# Autodesk Inventor assembly: Ensamblaje del tambor con sis. Lebus
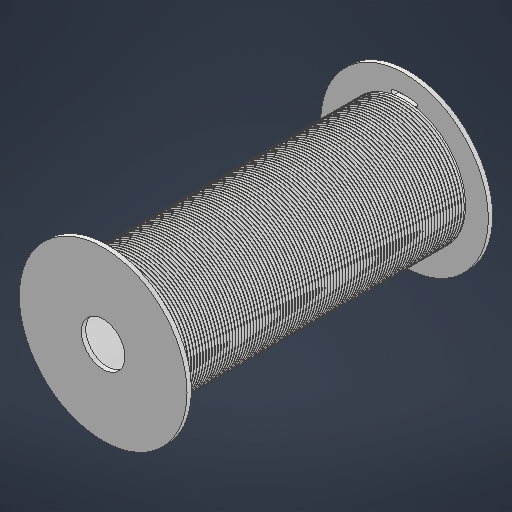
[picture p0: Inventor's stored thumbnail of the model, 512x512]
Saved by Autodesk Inventor 2026 (Build 300175050, 175E)
## iProperties
Created: 2025-07-06
Part Number: Ensamblaje del tambor con sis. Lebus
Document SubType Name: Conjunto soldado
Designer: Daniel Rodriguez
Weld Material: Genérico
Author: Daniel Rodriguez
## Documents named in this file (5)
- C:\Users\Daniel Rodriguez\Downloads\winch-drum-welding-assembly\Nuestro Winch\Sistema LEBUS\Ensamblaje del tambor con sis. Lebus.iam
- C:\Users\Daniel Rodriguez\Downloads\winch-drum-welding-assembly\Nuestro Winch\Sistema LEBUS\Tambor liso (drum).ipt
- C:\Users\Daniel Rodriguez\Downloads\winch-drum-welding-assembly\Nuestro Winch\Sistema LEBUS\Sistema LEBUS.ipt
- C:\Users\Daniel Rodriguez\Downloads\winch-drum-welding-assembly\Nuestro Winch\Sistema LEBUS\Brida_1 (flange_1) Lebus.ipt
- C:\Users\Daniel Rodriguez\Downloads\winch-drum-welding-assembly\Nuestro Winch\Sistema LEBUS\Brida_2 (flange_2) Lebus.ipt
## Components (4 placed, 4 different names)
1. Tambor liso (drum):1 — Coincidencia:1, Coincidencia:2, Coincidencia:3, Insertar:1, Insertar:2
2. Sistema LEBUS:1 — Coincidencia:2, Coincidencia:3
3. Brida_1 (flange_1) Lebus:1 — Insertar:1
4. Brida_2 (flange_2) Lebus:1 — Insertar:2
## Relationships (5: Mate 3, Insert 2)
- Coincidencia:1 [Mate]: Tambor liso (drum):1
- Coincidencia:2 [Mate]: Tambor liso (drum):1 ↔ Sistema LEBUS:1
- Coincidencia:3 [Mate]: Tambor liso (drum):1 ↔ Sistema LEBUS:1
- Insertar:1: Tambor liso (drum):1 ↔ Brida_1 (flange_1) Lebus:1
- Insertar:2: Tambor liso (drum):1 ↔ Brida_2 (flange_2) Lebus:1
